# Autodesk Inventor assembly: Compressor 1764
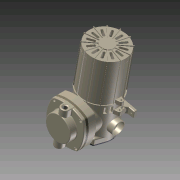
[picture p0: Inventor's stored thumbnail of the model, 180x180]
Saved by Autodesk Inventor 2011 (Build 150239000, 239)
## iProperties
Created: 2010-01-18
Part Number: Compressor 1764
Document SubType Name: Assembly
Designer: wbridges
Author: wbridges
## Documents named in this file (10)
- R:\CAD Archives\Pnewmatics\Compressor 1764\Compressor 1764.iam
- R:\CAD Archives\Pnewmatics\Compressor 1764\Between Seal 1764.ipt
- R:\CAD Archives\Pnewmatics\Compressor 1764\Top Cap 1764.ipt
- R:\CAD Archives\Pnewmatics\Compressor 1764\O-Ring 1764.ipt
- R:\CAD Archives\Pnewmatics\Compressor 1764\Metal Cylinder Seal 1764.ipt
- R:\CAD Archives\Pnewmatics\Compressor 1764\Top Part 1764.ipt
- R:\CAD Archives\Pnewmatics\Compressor 1764\Compressor Frame 1764.ipt
- R:\CAD Archives\Pnewmatics\Compressor 1764\Top Part Cap 1764.ipt
- R:\CAD Archives\Pnewmatics\Compressor 1764\Back Plate 1764.ipt
- R:\CAD Archives\Pnewmatics\Compressor 1764\Back Plate 2 1764.ipt
## Components (9 placed, 9 different names)
1. Between Seal 1764:1 — Mate:1, Mate:2, Mate:3, Mate:4, Tangent:1, Mate:5, Mate:8, Mate:9, Mate:10
2. Top Cap 1764:1 — Mate:8, Mate:9, Mate:10
3. O-Ring 1764:1 — Mate:4, Tangent:1, Tangent:2
4. Metal Cylinder Seal 1764:1 — Mate:5, Tangent:2
5. Top Part 1764:1 — Mate:6, Mate:7, Mate:11, Mate:12, Flush:1, Flush:2
6. Compressor Frame 1764:1 — Mate:1, Mate:2, Mate:3, Mate:6, Mate:7, Mate:11, Mate:13, Mate:14, Mate:15
7. Top Part Cap 1764:1 — Mate:12, Flush:1, Flush:2
8. Back Plate 1764:1 — Mate:16, Mate:17, Mate:18
9. Back Plate 2 1764:1 — Mate:13, Mate:14, Mate:15, Mate:16, Mate:17, Mate:18
## Relationships (22: Mate 18, Tangent 2, Flush 2)
- Mate:1: Between Seal 1764:1 ↔ Compressor Frame 1764:1
- Mate:2: Between Seal 1764:1 ↔ Compressor Frame 1764:1
- Mate:3: Between Seal 1764:1 ↔ Compressor Frame 1764:1
- Mate:4: Between Seal 1764:1 ↔ O-Ring 1764:1
- Tangent:1: Between Seal 1764:1 ↔ O-Ring 1764:1
- Mate:5: Between Seal 1764:1 ↔ Metal Cylinder Seal 1764:1
- Tangent:2: O-Ring 1764:1 ↔ Metal Cylinder Seal 1764:1
- Mate:6: Top Part 1764:1 ↔ Compressor Frame 1764:1
- Mate:7: Top Part 1764:1 ↔ Compressor Frame 1764:1
- Mate:8: Between Seal 1764:1 ↔ Top Cap 1764:1
- Mate:9: Between Seal 1764:1 ↔ Top Cap 1764:1
- Mate:10: Between Seal 1764:1 ↔ Top Cap 1764:1
- Mate:11: Top Part 1764:1 ↔ Compressor Frame 1764:1
- Mate:12: Top Part 1764:1 ↔ Top Part Cap 1764:1
- Flush:1: Top Part 1764:1 ↔ Top Part Cap 1764:1
- Flush:2: Top Part 1764:1 ↔ Top Part Cap 1764:1
- Mate:13: Compressor Frame 1764:1 ↔ Back Plate 2 1764:1
- Mate:14: Compressor Frame 1764:1 ↔ Back Plate 2 1764:1
- Mate:15: Compressor Frame 1764:1 ↔ Back Plate 2 1764:1
- Mate:16: Back Plate 1764:1 ↔ Back Plate 2 1764:1
- Mate:17: Back Plate 1764:1 ↔ Back Plate 2 1764:1
- Mate:18: Back Plate 1764:1 ↔ Back Plate 2 1764:1
